# Autodesk Inventor assembly: Chassis
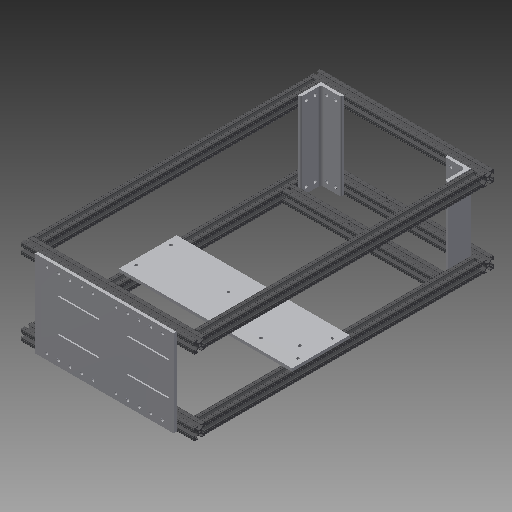
[picture p0: Inventor's stored thumbnail of the model, 512x512]
Saved by Autodesk Inventor 2017 SP1 (Build 210196100, 196)
## iProperties
Created: 2016-04-02
Part Number: Chassis
Document SubType Name: Assembly
Designer: hwasserb
Author: hwasserb
## Documents named in this file (10)
- C:\Users\Haden\Desktop\Charlie-CAD-Model\Robot Model\Chassis\Chassis.iam
- C:\Users\Haden\Desktop\Charlie-CAD-Model\Robot Model\Chassis\Front Bar.ipt
- C:\Users\Haden\Desktop\Charlie-CAD-Model\Robot Model\Chassis\Long Bar Upper.ipt
- C:\Users\Haden\Desktop\Charlie-CAD-Model\Robot Model\Chassis\Back Bar Upper.ipt
- C:\Users\Haden\Desktop\Charlie-CAD-Model\Robot Model\Chassis\Right Angle.ipt
- C:\Users\Haden\Desktop\Charlie-CAD-Model\Robot Model\Chassis\Long Bar Lower.ipt
- C:\Users\Haden\Desktop\Charlie-CAD-Model\Robot Model\Chassis\Back Bar Lower.ipt
- C:\Users\Haden\Desktop\Charlie-CAD-Model\Robot Model\Chassis\Wheel Support.ipt
- C:\Users\Haden\Desktop\Charlie-CAD-Model\Robot Model\Chassis\Power Panel.ipt
- C:\Users\Haden\Desktop\Charlie-CAD-Model\Robot Model\Chassis\LiDAR Plate.ipt
## Components (13 placed, 9 different names)
1. Front Bar:1 — Flush:1, Flush:2, Mate:32, Mate:33, Mate:50, Mate:51, Mate:52, Mate:53, Mate:54, Mate:55, Mate:56, Mate:57, Mate:58, Mate:59
2. Front Bar:2 — Flush:1, Flush:2, Mate:1, Mate:2, Flush:3, Flush:4, Mate:3, Mate:4, Mate:39, Mate:40, Mate:41, Mate:42, Mate:43, Mate:44, Mate:45, Mate:46, Mate:47, Mate:48, Mate:49
3. Long Bar Upper:1 — Mate:1, Flush:3, Mate:4, Mate:5, Mate:7, Mate:14, Mate:15
4. Long Bar Upper:2 — Mate:2, Flush:4, Mate:3, Mate:6, Mate:8, Mate:9
5. Back Bar Upper:1 — Mate:5, Mate:6, Mate:7, Mate:10, Mate:11, Mate:12, Mate:13
6. Right Angle:1 — Mate:8, Mate:9, Mate:10, Mate:11, Mate:18, Mate:19, Mate:20, Mate:26, Mate:27
7. Right Angle:2 — Mate:12, Mate:13, Mate:14, Mate:15, Mate:16, Mate:17, Mate:21, Mate:24, Mate:25
8. Long Bar Lower:1 — Mate:16, Mate:17, Mate:21, Mate:22, Mate:23, Mate:29, Flush:5, Mate:30, Mate:32, Mate:34, Mate:37, Mate:38
9. Long Bar Lower:2 — Mate:18, Mate:19, Mate:20, Mate:28, Mate:31, Mate:33, Mate:35, Mate:36
10. Back Bar Lower:1 — Mate:22, Mate:23, Mate:24, Mate:25, Mate:26, Mate:27, Mate:28
11. Wheel Support:1 — Mate:29, Flush:5, Mate:30, Mate:31
12. Power Panel:1 — Mate:34, Mate:35, Mate:36, Mate:37, Mate:38
13. LiDAR Plate:1 — Mate:39, Mate:40, Mate:41, Mate:42, Mate:43, Mate:44, Mate:45, Mate:46, Mate:47, Mate:48, Mate:49, Mate:50, Mate:51, Mate:52, Mate:53, Mate:54, Mate:55, Mate:56, Mate:57, Mate:58, Mate:59
## Relationships (64: Mate 59, Flush 5)
- Flush:1: Front Bar:1 ↔ Front Bar:2
- Flush:2: Front Bar:1 ↔ Front Bar:2
- Mate:1: Front Bar:2 ↔ Long Bar Upper:1
- Mate:2: Front Bar:2 ↔ Long Bar Upper:2
- Flush:3: Front Bar:2 ↔ Long Bar Upper:1
- Flush:4: Front Bar:2 ↔ Long Bar Upper:2
- Mate:3: Front Bar:2 ↔ Long Bar Upper:2
- Mate:4: Front Bar:2 ↔ Long Bar Upper:1
- Mate:5: Long Bar Upper:1 ↔ Back Bar Upper:1
- Mate:6: Long Bar Upper:2 ↔ Back Bar Upper:1
- Mate:7: Long Bar Upper:1 ↔ Back Bar Upper:1
- Mate:8: Long Bar Upper:2 ↔ Right Angle:1
- Mate:9: Long Bar Upper:2 ↔ Right Angle:1
- Mate:10: Back Bar Upper:1 ↔ Right Angle:1
- Mate:11: Back Bar Upper:1 ↔ Right Angle:1
- Mate:12: Back Bar Upper:1 ↔ Right Angle:2
- Mate:13: Back Bar Upper:1 ↔ Right Angle:2
- Mate:14: Long Bar Upper:1 ↔ Right Angle:2
- Mate:15: Long Bar Upper:1 ↔ Right Angle:2
- Mate:16: Right Angle:2 ↔ Long Bar Lower:1
- Mate:17: Right Angle:2 ↔ Long Bar Lower:1
- Mate:18: Right Angle:1 ↔ Long Bar Lower:2
- Mate:19: Right Angle:1 ↔ Long Bar Lower:2
- Mate:20: Right Angle:1 ↔ Long Bar Lower:2
- Mate:21: Right Angle:2 ↔ Long Bar Lower:1
- Mate:22: Long Bar Lower:1 ↔ Back Bar Lower:1
- Mate:23: Long Bar Lower:1 ↔ Back Bar Lower:1
- Mate:24: Right Angle:2 ↔ Back Bar Lower:1
- Mate:25: Right Angle:2 ↔ Back Bar Lower:1
- Mate:26: Right Angle:1 ↔ Back Bar Lower:1
- Mate:27: Right Angle:1 ↔ Back Bar Lower:1
- Mate:28: Long Bar Lower:2 ↔ Back Bar Lower:1
- Mate:29: Long Bar Lower:1 ↔ Wheel Support:1
- Flush:5: Long Bar Lower:1 ↔ Wheel Support:1
- Mate:30: Long Bar Lower:1 ↔ Wheel Support:1
- Mate:31: Long Bar Lower:2 ↔ Wheel Support:1
- Mate:32: Front Bar:1 ↔ Long Bar Lower:1
- Mate:33: Front Bar:1 ↔ Long Bar Lower:2
- Mate:34: Long Bar Lower:1 ↔ Power Panel:1
- Mate:35: Long Bar Lower:2 ↔ Power Panel:1
- Mate:36: Long Bar Lower:2 ↔ Power Panel:1
- Mate:37: Long Bar Lower:1 ↔ Power Panel:1
- Mate:38: Long Bar Lower:1 ↔ Power Panel:1
- Mate:39: Front Bar:2 ↔ LiDAR Plate:1
- Mate:40: Front Bar:2 ↔ LiDAR Plate:1
- Mate:41: Front Bar:2 ↔ LiDAR Plate:1
- Mate:42: Front Bar:2 ↔ LiDAR Plate:1
- Mate:43: Front Bar:2 ↔ LiDAR Plate:1
- Mate:44: Front Bar:2 ↔ LiDAR Plate:1
- Mate:45: Front Bar:2 ↔ LiDAR Plate:1
- Mate:46: Front Bar:2 ↔ LiDAR Plate:1
- Mate:47: Front Bar:2 ↔ LiDAR Plate:1
- Mate:48: Front Bar:2 ↔ LiDAR Plate:1
- Mate:49: Front Bar:2 ↔ LiDAR Plate:1
- Mate:50: Front Bar:1 ↔ LiDAR Plate:1
- Mate:51: Front Bar:1 ↔ LiDAR Plate:1
- Mate:52: Front Bar:1 ↔ LiDAR Plate:1
- Mate:53: Front Bar:1 ↔ LiDAR Plate:1
- Mate:54: Front Bar:1 ↔ LiDAR Plate:1
- Mate:55: Front Bar:1 ↔ LiDAR Plate:1
- Mate:56: Front Bar:1 ↔ LiDAR Plate:1
- Mate:57: Front Bar:1 ↔ LiDAR Plate:1
- Mate:58: Front Bar:1 ↔ LiDAR Plate:1
- Mate:59: Front Bar:1 ↔ LiDAR Plate:1
